# Autodesk Inventor assembly: F-Upright2018
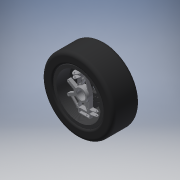
[picture p0: Inventor's stored thumbnail of the model, 180x180]
Saved by Autodesk Inventor 2018.2 (Build 222227000, 227)
## iProperties
Created: 2018-05-19
Part Number: F-Upright2018
Material: 一般
Document SubType Name: Assembly
Designer: ku_sk
Sending System: Autodesk Inventor 2018
Preprocessor: ST-DEVELOPER v17
Title: D:\ku_sk\ドキュメント\Inventor\Aero\KS-15\全体アッセンブリ解析用モデル\body\sus\F-Upright2018.stp
Author: ku_sk
## Documents named in this file (5)
- D:\ku_sk\ドキュメント\Inventor\Aero\KS-15\全体アッセンブリ解析用モデル\body\sus\F-Upright2018.iam
- D:\ku_sk\ドキュメント\Inventor\Aero\KS-15\全体アッセンブリ解析用モデル\body\sus\Part3.ipt
- D:\ku_sk\ドキュメント\Inventor\Aero\KS-15\全体アッセンブリ解析用モデル\body\sus\Part4.ipt
- D:\ku_sk\ドキュメント\Inventor\Aero\KS-15\全体アッセンブリ解析用モデル\body\sus\Part2.ipt
- D:\ku_sk\ドキュメント\Inventor\Aero\KS-15\全体アッセンブリ解析用モデル\body\sus\2015Wheel watanabe.ipt
## Components (4 placed, 4 different names)
1. Part3.1 — メイト:1, メイト:2
2. Part4.1
3. Part2.1
4. 2015Wheel watanabe:1 — メイト:1, メイト:2
## Relationships (2: Mate 2)
- メイト:1 [Mate]: Part3.1 ↔ 2015Wheel watanabe:1
- メイト:2 [Mate] (49 mm): Part3.1 ↔ 2015Wheel watanabe:1
